# Autodesk Inventor assembly: traction_wheel_MIR
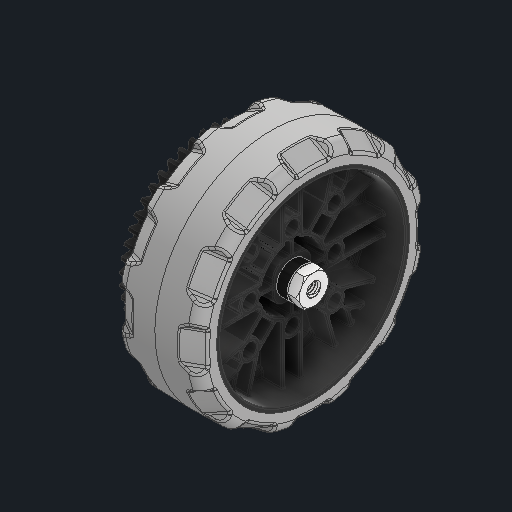
[picture p0: Inventor's stored thumbnail of the model, 512x512]
Saved by Autodesk Inventor 2024 (Build 280153000, 153)
## iProperties
Created: 2023-10-18
Part Number: traction_wheel_MIR
Document SubType Name: Assembly
Designer: Averey Ku
Author: Averey Ku
## Documents named in this file (7)
- D:\vex_robotics\hardware\cad\goated_v0.1\chassis\mirrored_parts\traction_wheel_MIR.iam
- D:\vex_robotics\hardware\cad\VEX-CAD-Inventor-1.41\Structure\Hardware\Nut Nylon\Nut Nylon - White.ipt
- D:\vex_robotics\hardware\cad\VEX-CAD-Inventor-1.41\Structure\Hardware\Nut Nylon.ipt
- D:\vex_robotics\hardware\cad\VEX-CAD-Inventor-1.41\Motion\Spacers\Spacer Nylon .375 OD\NSpacer .375 OD x .125.ipt
- D:\vex_robotics\hardware\cad\VEX-CAD-Inventor-1.41\Motion\Spacers\Spacer Nylon .375 OD.ipt
- D:\vex_robotics\hardware\cad\goated_v0.1\chassis\mirrored_parts\2.75 Traction AS, No Insert_MIR.iam
- D:\vex_robotics\hardware\cad\goated_v0.1\chassis\mirrored_parts\ls_48t_MIR.ipt
## Components (4 placed, 4 different names)
1. Nut Nylon - White:1 — Insert:1
2. NSpacer .375 OD x .125:1 — Insert:1, Insert:3
3. 2.75 Traction AS, No Insert_MIR:1 [sub-assembly] — Insert:3, Insert:2
4. ls_48t_MIR:1 — Insert:2
## Relationships (3: Insert 3)
- Insert:1: Nut Nylon - White:1 ↔ NSpacer .375 OD x .125:1
- Insert:3: NSpacer .375 OD x .125:1 ↔ 2.75 Traction AS, No Insert_MIR:1
- Insert:2 (3.175 mm): 2.75 Traction AS, No Insert_MIR:1 ↔ ls_48t_MIR:1
